# Autodesk Inventor assembly: Motor arm assembly final
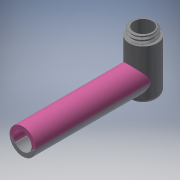
[picture p0: Inventor's stored thumbnail of the model, 180x180]
Saved by Autodesk Inventor 2019 (Build 230136000, 136)
## iProperties
Created: 2020-03-26
Part Number: Motor arm assembly final
Document SubType Name: Assembly
Designer: 18186
Author: 18186
## Documents named in this file (4)
- D:\CoDrone\Motor arm assembly final.iam
- D:\CoDrone\drone motor arm bottom.ipt
- D:\CoDrone\drone motor arm top.ipt
- D:\CoDrone\Part1.ipt
## Components (3 placed, 3 different names)
1. drone motor arm bottom:1 — Mate:1, Flush:1, Flush:2
2. drone motor arm top:1 — Mate:1, Flush:1
3. Part1:1 — Flush:2
## Relationships (3: Flush 2, Mate 1)
- Mate:1: drone motor arm bottom:1 ↔ drone motor arm top:1
- Flush:1: drone motor arm bottom:1 ↔ drone motor arm top:1
- Flush:2: drone motor arm bottom:1 ↔ Part1:1
